# Autodesk Inventor assembly: Assembly_Cube_Z_stage_sample_outercube_motorized
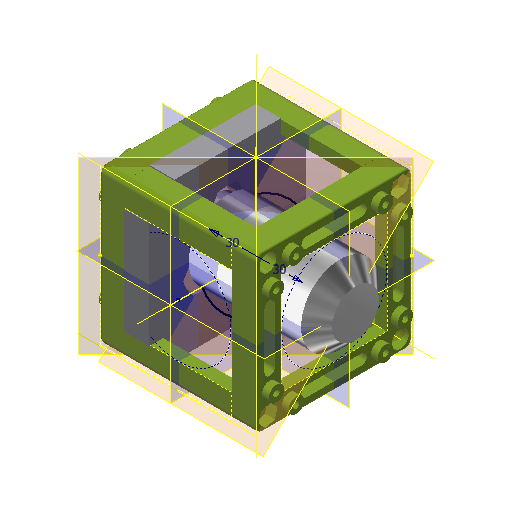
[picture p0: Inventor's stored thumbnail of the model, 512x512]
Saved by Autodesk Inventor 2022 (Build 260153000, 153)
## iProperties
Created: 2020-10-26
Part Number: Assembly_Cube_Z_stage_sample_outercube_motorized
Document SubType Name: Assembly
Designer: diederichbenedict
Author: diederichbenedict
## Documents named in this file (4)
- C:\Users\PrakashLab\Documents\UC2-INVENTOR-Git\uc2_v3\Assembly_Cube_RMS_objective.iam
- C:\Users\PrakashLab\Documents\UC2-INVENTOR-Git\uc2_v3\00_Microscope_Objective_Lens10x.ipt
- C:\Users\PrakashLab\Documents\UC2-INVENTOR-Git\uc2_v3\Assembly_Cube_empty_IM_v3.iam
- C:\Users\PrakashLab\Documents\UC2-INVENTOR-Git\uc2_v3\20_Cube_Insert_Lens_holder_RMS_63x.ipt
## Components (3 placed, 3 different names)
1. Assembly_Cube_empty_IM_v3:1 [sub-assembly] — Mate:2, Mate:3
2. 20_Cube_Insert_Lens_holder_RMS_63x:1 — Insert:1, Mate:3
3. 00_Microscope_Objective_Lens10x:1 — Insert:1, Mate:2
## Relationships (5: Mate 3, Angle 1, Insert 1)
- [Mate]: Assembly_Cube_empty_IM_v3:1 ↔ 20_Cube_Insert_Lens_holder_RMS_63x:1
- [Angle] (0 deg): Assembly_Cube_empty_IM_v3:1 ↔ 20_Cube_Insert_Lens_holder_RMS_63x:1
- Insert:1: 20_Cube_Insert_Lens_holder_RMS_63x:1 ↔ 00_Microscope_Objective_Lens10x:1
- Mate:2: Assembly_Cube_empty_IM_v3:1 ↔ 00_Microscope_Objective_Lens10x:1
- Mate:3: Assembly_Cube_empty_IM_v3:1 ↔ 20_Cube_Insert_Lens_holder_RMS_63x:1
